# Autodesk Inventor assembly: DHT_sestava
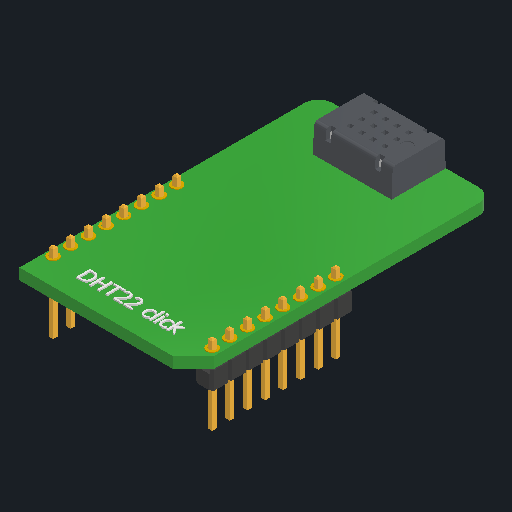
[picture p0: Inventor's stored thumbnail of the model, 512x512]
Saved by Autodesk Inventor 2022 (Build 260153000, 153)
## iProperties
Created: 2022-03-19
Part Number: DHT_sestava
Document SubType Name: Assembly
Designer: dvorakj
Author: dvorakj
## Documents named in this file (4)
- C:\Users\dvorakj\Documents\Inventor\Bakalarka\Clicks\DHT22\DHT_sestava.iam
- C:\Users\dvorakj\Documents\Inventor\Bakalarka\Clicks\DHT22\DHT22_pcb.ipt
- C:\Users\dvorakj\Documents\Inventor\Bakalarka\Clicks\Pin Header\61300811121 (rev1).iam
- C:\Users\dvorakj\Documents\Inventor\Bakalarka\Clicks\DHT22\Senzor\AM2322.ipt
## Components (4 placed, 3 different names)
1. DHT22_pcb:1 — Mate:1, Mate:2, Mate:3, Mate:4, Mate:5
2. 61300811121 (rev1):1 [sub-assembly] — Mate:2, Mate:4
3. 61300811121 (rev1):2 [sub-assembly] — Mate:1, Mate:3
4. AM2322:1 — Mate:5
## Relationships (5: Mate 5)
- Mate:1: DHT22_pcb:1 ↔ 61300811121 (rev1):2
- Mate:2: DHT22_pcb:1 ↔ 61300811121 (rev1):1
- Mate:3: DHT22_pcb:1 ↔ 61300811121 (rev1):2
- Mate:4: DHT22_pcb:1 ↔ 61300811121 (rev1):1
- Mate:5: DHT22_pcb:1 ↔ AM2322:1
